# Autodesk Inventor assembly: semifinal
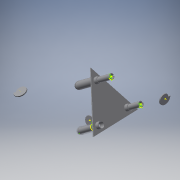
[picture p0: Inventor's stored thumbnail of the model, 180x180]
Saved by Autodesk Inventor 2018 (Build 220112000, 112)
## iProperties
Created: 2019-05-27
Part Number: semifinal
Document SubType Name: Assembly
Designer: Piyush
Author: Piyush
## Documents named in this file (6)
- C:\Users\Piyush\Documents\semifinal.iam
- C:\Users\Piyush\Documents\base1.ipt
- C:\Users\Piyush\Documents\guide1.ipt
- C:\Users\Piyush\Documents\pusher.ipt
- C:\Users\Piyush\Documents\leg.iam
- C:\Users\Piyush\Documents\camn.ipt
## Components (13 placed, 5 different names)
1. base1:1 — Mate:1, Rotational:1, Rotational:2, Rotational:3, Rotational:4, Rotational:5, Rotational:6
2. guide1:1 — Rotational:1, Mate:2
3. guide1:2 — Rotational:3, Mate:4
4. guide1:3 — Rotational:2, Mate:3
5. pusher:1 — Mate:1, Mate:2
6. pusher:2 — Mate:3, Mate:6, Mate:7, Mate:8
7. pusher:3 — Mate:4
8. leg:1 [sub-assembly] — Rotational:4
9. leg:2 [sub-assembly] — Rotational:6
10. leg:3 [sub-assembly] — Rotational:5
11. camn:1
12. camn:2 — Mate:6, Mate:7, Mate:8
13. camn:3
## Relationships (13: Mate 7, RevoluteJoint 6)
- Mate:1: base1:1 ↔ pusher:1
- Rotational:1 [RevoluteJoint]: base1:1 ↔ guide1:1
- Rotational:2 [RevoluteJoint]: base1:1 ↔ guide1:3
- Rotational:3 [RevoluteJoint]: base1:1 ↔ guide1:2
- Mate:2: guide1:1 ↔ pusher:1
- Mate:3: guide1:3 ↔ pusher:2
- Mate:4: guide1:2 ↔ pusher:3
- Rotational:4 [RevoluteJoint]: base1:1 ↔ leg:1
- Rotational:5 [RevoluteJoint]: base1:1 ↔ leg:3
- Rotational:6 [RevoluteJoint]: base1:1 ↔ leg:2
- Mate:6: pusher:2 ↔ camn:2
- Mate:7 (31.25 mm): pusher:2 ↔ camn:2
- Mate:8 (31.25 mm): pusher:2 ↔ camn:2
